# Autodesk Inventor assembly: pootbeen3
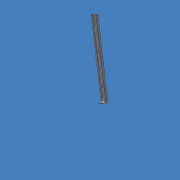
[picture p0: Inventor's stored thumbnail of the model, 180x180]
Saved by Autodesk Inventor 2015 (Build 190159000, 159)
## iProperties
Created: 2007-07-03
Part Number: pootbeen3
Document SubType Name: Assembly
Designer: kurt
Manufacturer: Standard
Standards Organization: Custom
Author: kurt
## Documents named in this file (3)
- F:\Tekeningen\bibliotheek\poten\Sub-assemblys\90-10-0950.iam
- F:\Tekeningen\bibliotheek\poten\onderdelen\90-07-0950.ipt
- F:\Tekeningen\bibliotheek\poten\onderdelen\90-01-0000.ipt
## Components (2 placed, 2 different names)
1. 90-07-0950:1 — Mate:1, Mate:2, Mate:3
2. 90-01-0000:1 — Mate:1, Mate:2, Mate:3
## Relationships (3: Mate 3)
- Mate:1: 90-07-0950:1 ↔ 90-01-0000:1
- Mate:2: 90-07-0950:1 ↔ 90-01-0000:1
- Mate:3: 90-07-0950:1 ↔ 90-01-0000:1
